# Autodesk Inventor assembly: SUSPENSION UNIT_MIR
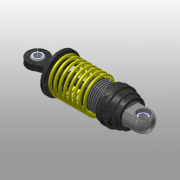
[picture p0: Inventor's stored thumbnail of the model, 180x180]
Saved by Autodesk Inventor 2015 (Build 190159000, 159)
## iProperties
Created: 2015-04-18
Part Number: SUSPENSION UNIT_MIR
Document SubType Name: Assembly
Designer: Station9
Author: Station9
## Documents named in this file (10)
- D:\Project Archive\AD\AD-6(94.01.29)WSC2011\SUSPENSION UNIT_MIR.iam
- D:\Project Archive\AD\AD-6(94.01.29)WSC2011\500-102_MIR.ipt
- D:\Project Archive\AD\AD-6(94.01.29)WSC2011\500-106_MIR.ipt
- D:\Project Archive\AD\AD-6(94.01.29)WSC2011\500-105_MIR.ipt
- D:\Project Archive\AD\AD-6(94.01.29)WSC2011\500-109_MIR.ipt
- D:\Project Archive\AD\AD-6(94.01.29)WSC2011\500-104_MIR.ipt
- D:\Project Archive\AD\AD-6(94.01.29)WSC2011\500-103_MIR.ipt
- D:\Project Archive\AD\AD-6(94.01.29)WSC2011\500-100_MIR.ipt
- D:\Project Archive\AD\AD-6(94.01.29)WSC2011\Compression Spring 16_MIR.ipt
- D:\Project Archive\AD\AD-6(94.01.29)WSC2011\500-107_MIR.ipt
## Components (10 placed, 9 different names)
1. 500-102_MIR:1 — Mate:9, Mate:13
2. 500-106_MIR:1 — Mate:6, Flush:1, Angle:3, Mate:12, Mate:15
3. 500-105_MIR:1 — Insert:1, Mate:4, Mate:3
4. 500-109_MIR:1 — Angle:2, Mate:2, Mate:1
5. 500-104_MIR:1 — Mate:9, Mate:6, Mate:11, Mate:5, Mate:8, Mate:14
6. 500-103_MIR:1 — Mate:11, Angle:2, Mate:5, Insert:1, Mate:2, Mate:1
7. 500-100_MIR:1 — Mate:13, Flush:1, Mate:8
8. Compression Spring 16_MIR:1 — Mate:4, Mate:3
9. 500-109_MIR:2 — Angle:3, Mate:12
10. 500-107_MIR:1 — Mate:15, Mate:14
## Relationships (17: Mate 13, Angle 2, Insert 1, Flush 1)
- Mate:9: 500-102_MIR:1 ↔ 500-104_MIR:1
- Mate:6: 500-106_MIR:1 ↔ 500-104_MIR:1
- Mate:11: 500-104_MIR:1 ↔ 500-103_MIR:1
- Angle:2 (0 deg): 500-109_MIR:1 ↔ 500-103_MIR:1
- Mate:5: 500-104_MIR:1 ↔ 500-103_MIR:1
- Insert:1: 500-105_MIR:1 ↔ 500-103_MIR:1
- Mate:2: 500-109_MIR:1 ↔ 500-103_MIR:1
- Mate:1: 500-109_MIR:1 ↔ 500-103_MIR:1
- Mate:13: 500-102_MIR:1 ↔ 500-100_MIR:1
- Flush:1: 500-106_MIR:1 ↔ 500-100_MIR:1
- Mate:8: 500-104_MIR:1 ↔ 500-100_MIR:1
- Mate:4: 500-105_MIR:1 ↔ Compression Spring 16_MIR:1
- Mate:3: 500-105_MIR:1 ↔ Compression Spring 16_MIR:1
- Angle:3 (0 deg): 500-106_MIR:1 ↔ 500-109_MIR:2
- Mate:12: 500-106_MIR:1 ↔ 500-109_MIR:2
- Mate:15: 500-106_MIR:1 ↔ 500-107_MIR:1
- Mate:14: 500-104_MIR:1 ↔ 500-107_MIR:1
